# Autodesk Inventor assembly: цепь_MIR1
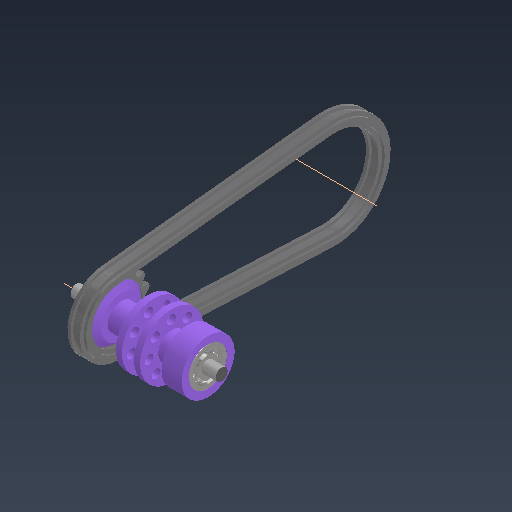
[picture p0: Inventor's stored thumbnail of the model, 512x512]
Saved by Autodesk Inventor 2025.2 (Build 292293000, 293)
## iProperties
Created: 2024-07-09
Part Number: цепь_MIR1
Document SubType Name: Assembly
Designer: Trene
Author: Phantom
## Documents named in this file (6)
- F:\Phantom16950-main\цепь_MIR1.iam
- F:\Phantom16950-main\Цепной привод2_MIR1.iam
- F:\Phantom16950-main\втулка для подш 2 часть_MIR3.ipt
- F:\Phantom16950-main\втулка для подш_MIR3.ipt
- F:\Phantom16950-main\Деталь_64_MIR3.ipt
- F:\Phantom16950-main\BS 290 SKF - SKF 626-RZ_MIR3.ipt
## Components (6 placed, 5 different names)
1. Цепной привод2_MIR1:1 [sub-assembly] — Заподлицо:4, Совмещение:24, Совмещение:22
2. втулка для подш 2 часть_MIR3:1 — Совмещение:16, Совмещение:23, Совмещение:20
3. втулка для подш_MIR3:1 — Заподлицо:4, Совмещение:24, Совмещение:22, Совмещение:16, Совмещение:17, Совмещение:18
4. Деталь_64_MIR3:1 — Совмещение:23, Совмещение:17, Совмещение:21, Совмещение:19
5. BS 290 SKF - SKF 626-RZ_MIR3:1 — Совмещение:21, Совмещение:20
6. BS 290 SKF - SKF 626-RZ_MIR3:2 — Совмещение:19, Совмещение:18
## Relationships (10: Mate 9, Flush 1)
- Заподлицо:4 [Flush] (4 mm): Цепной привод2_MIR1:1 ↔ втулка для подш_MIR3:1
- Совмещение:24 [Mate]: Цепной привод2_MIR1:1 ↔ втулка для подш_MIR3:1
- Совмещение:22 [Mate]: Цепной привод2_MIR1:1 ↔ втулка для подш_MIR3:1
- Совмещение:16 [Mate]: втулка для подш 2 часть_MIR3:1 ↔ втулка для подш_MIR3:1
- Совмещение:23 [Mate]: втулка для подш 2 часть_MIR3:1 ↔ Деталь_64_MIR3:1
- Совмещение:17 [Mate]: втулка для подш_MIR3:1 ↔ Деталь_64_MIR3:1
- Совмещение:21 [Mate]: Деталь_64_MIR3:1 ↔ BS 290 SKF - SKF 626-RZ_MIR3:1
- Совмещение:20 [Mate]: втулка для подш 2 часть_MIR3:1 ↔ BS 290 SKF - SKF 626-RZ_MIR3:1
- Совмещение:19 [Mate]: Деталь_64_MIR3:1 ↔ BS 290 SKF - SKF 626-RZ_MIR3:2
- Совмещение:18 [Mate]: втулка для подш_MIR3:1 ↔ BS 290 SKF - SKF 626-RZ_MIR3:2
